# Autodesk Inventor assembly: canard_assemb2
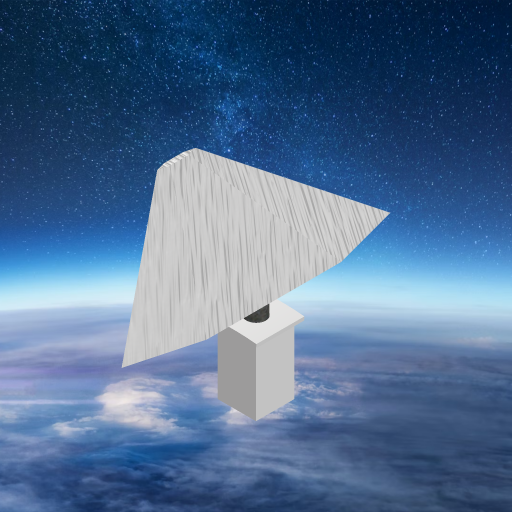
[picture p0: Inventor's stored thumbnail of the model, 512x512]
Saved by Autodesk Inventor 2023 (Build 270158000, 158)
## iProperties
Created: 2023-10-24
Part Number: canard_assemb2
Document SubType Name: Assembly
Designer: 310611102
Author: 310611102
## Documents named in this file (4)
- C:\Users\310611102\Documents\Inventor\SSR\avionics_2023ver\assembly\canard_assemb2.iam
- C:\Users\310611102\Documents\Inventor\SSR\avionics_2023ver\actuator_system\shiftt_fixed_plate.ipt
- C:\Users\310611102\Documents\Inventor\SSR\avionics_2023ver\actuator_system\gearbox_temp\gearbox_shaft3.ipt
- C:\Users\310611102\Documents\Inventor\SSR\avionics_2023ver\actuator_system\canard.ipt
## Components (3 placed, 3 different names)
1. shiftt_fixed_plate:1 — Insert:1
2. gearbox_shaft3:1 — Insert:1, Insert:2, Cylindrical:1
3. canard:1 — Insert:2, Cylindrical:1, Angle:1
## Relationships (4: Insert 2, CylindricalJoint 1, Angle 1)
- Insert:1: shiftt_fixed_plate:1 ↔ gearbox_shaft3:1
- Insert:2: gearbox_shaft3:1 ↔ canard:1
- Cylindrical:1: gearbox_shaft3:1 ↔ canard:1
- Angle:1 (180 deg): canard:1
